# Autodesk Inventor assembly: a板摆放
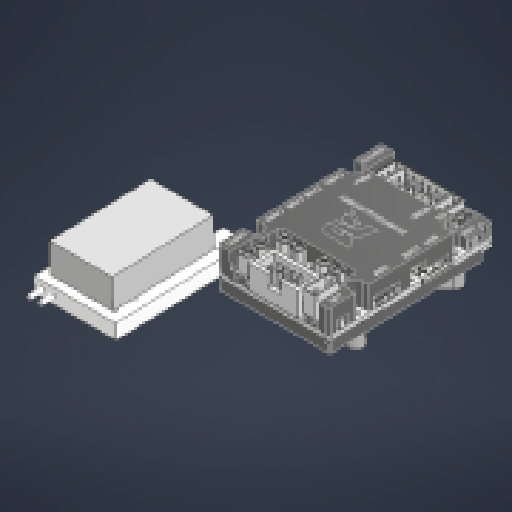
[picture p0: Inventor's stored thumbnail of the model, 512x512]
Saved by Autodesk Inventor 2025 (Build 290162000, 162)
## iProperties
Created: 2025-01-14
Part Number: a板摆放
Document SubType Name: Assembly
Designer: HZD
Author: HZD
## Documents named in this file (5)
- C:\1A_Engineering_files\GCG全向轮步兵\云台\a板摆放.iam
- C:\1A_Engineering_files\GCG全向轮步兵\云台\C型开发板.ipt
- C:\1A_Engineering_files\GCG全向轮步兵\云台\DR16接收机.ipt
- C:\1A_Engineering_files\GCG全向轮步兵\云台\C板辅助安装板.ipt
- C:\1A_Engineering_files\GCG全向轮步兵\云台\下载器.0002.ipt
## Components (4 placed, 4 different names)
1. C型开发板:1 — 配合:5, 配合:6, 配合:9, 表面齐平:1
2. DR16接收机:1 — 表面齐平:1
3. C板辅助安装板:1 — 配合:5, 配合:6, 配合:9
4. 下载器.0002:1
## Relationships (4: Mate 3, Flush 1)
- 配合:5 [Mate]: C型开发板:1 ↔ C板辅助安装板:1
- 配合:6 [Mate]: C型开发板:1 ↔ C板辅助安装板:1
- 配合:9 [Mate]: C型开发板:1 ↔ C板辅助安装板:1
- 表面齐平:1 [Flush]: C型开发板:1 ↔ DR16接收机:1
